# Autodesk Inventor assembly: modularRICH
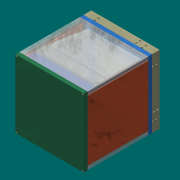
[picture p0: Inventor's stored thumbnail of the model, 180x180]
Saved by Autodesk Inventor 2016 (Build 200138000, 138)
## iProperties
Created: 2015-10-13
Part Number: modularRICH
Document SubType Name: Assembly
Designer: Sawaiz
Author: Sawaiz
## Documents named in this file (8)
- C:\Users\Sawaiz\OneDrive\projects\modularRICH\modularRICH.iam
- C:\Users\Sawaiz\OneDrive\projects\modularRICH\frame\frame.iam
- C:\Users\Sawaiz\OneDrive\projects\modularRICH\aerogelBlock.ipt
- C:\Users\Sawaiz\OneDrive\projects\modularRICH\fresnelLens.ipt
- C:\Users\Sawaiz\OneDrive\projects\modularRICH\mirror\mirrorTopBottom.ipt
- C:\Users\Sawaiz\OneDrive\projects\modularRICH\mirror\mirrorSides.ipt
- C:\Users\Sawaiz\OneDrive\projects\modularRICH\H12700A\H12700A.iam
- C:\Users\Sawaiz\OneDrive\projects\modularRICH\modularRICH.xlsx
## Components (8 placed, 6 different names)
1. frame:1 [sub-assembly] — Mate:1, Flush:1, Mate:3, Angle:4, Mate:4, Mate:5, Mate:6, Mate:7, Mate:8, Mate:9, Mate:10, Mate:11, Mate:12, Mate:13, Mate:14, Mate:15, Flush:3, Flush:4, Mate:16, Mate:17, Flush:5
2. aerogelBlock:1 — Mate:1, Flush:1, Mate:2, Mate:3
3. fresnelLens:1 — Mate:2, Flush:3, Flush:4
4. mirrorSides:1 — Angle:1, Mate:13, Mate:14, Mate:15
5. mirrorSides:2 — Angle:1, Angle:3, Mate:10, Mate:11, Mate:12
6. mirrorTopBottom:3 — Angle:2, Angle:3, Angle:4, Mate:4, Mate:5, Mate:6
7. mirrorTopBottom:4 — Angle:2, Mate:7, Mate:8, Mate:9
8. H12700A:1 [sub-assembly] — Mate:16, Mate:17, Flush:5
## Relationships (25: Mate 17, Flush 4, Angle 4)
- Mate:1: frame:1 ↔ aerogelBlock:1
- Flush:1 (6.35 mm): frame:1 ↔ aerogelBlock:1
- Mate:2: aerogelBlock:1 ↔ fresnelLens:1
- Mate:3: frame:1 ↔ aerogelBlock:1
- Angle:1 (180 deg): mirrorSides:1 ↔ mirrorSides:2
- Angle:2 (180 deg): mirrorTopBottom:3 ↔ mirrorTopBottom:4
- Angle:3 (90 deg): mirrorSides:2 ↔ mirrorTopBottom:3
- Angle:4 (180 deg): frame:1 ↔ mirrorTopBottom:3
- Mate:4: frame:1 ↔ mirrorTopBottom:3
- Mate:5: frame:1 ↔ mirrorTopBottom:3
- Mate:6: frame:1 ↔ mirrorTopBottom:3
- Mate:7: frame:1 ↔ mirrorTopBottom:4
- Mate:8: frame:1 ↔ mirrorTopBottom:4
- Mate:9: frame:1 ↔ mirrorTopBottom:4
- Mate:10: frame:1 ↔ mirrorSides:2
- Mate:11: frame:1 ↔ mirrorSides:2
- Mate:12 (-6.35 mm): frame:1 ↔ mirrorSides:2
- Mate:13: frame:1 ↔ mirrorSides:1
- Mate:14: frame:1 ↔ mirrorSides:1
- Mate:15 (-6.35 mm): frame:1 ↔ mirrorSides:1
- Flush:3 (3.175 mm): frame:1 ↔ fresnelLens:1
- Flush:4 (-3.175 mm): frame:1 ↔ fresnelLens:1
- Mate:16: frame:1 ↔ H12700A:1
- Mate:17: frame:1 ↔ H12700A:1
- Flush:5: frame:1 ↔ H12700A:1
## Named parameters: acrylicThickness = 6.35 mm, aerogelThickness = 20 mm, height = 101.6 mm, width = 101.6 mm, depth = 101.6 mm, mirrorAngle = 5 deg, detectorWidth = 52 mm, detectorHeight = 52 mm, mirrorThickness = 3 mm, fresnelThickness = 0.1 mm, grooveDensity = 100, focalLength = 76.2 mm, ior = 1.49, centerThickness = 1.524 mm, fresnelAngle = 90 deg, fresnelEffectiveDiameter = 76.2 mm, mirrorSuppourtWidth = 38.1 mm, backGrooveBit = 4.8006 mm, sensorHolderWidth = 88.9 mm, sensorHolderSesnorHeight = 53.975 mm, sensorHolderSensorWidth = 53.975 mm, sensorHolderHeight = 88.9 mm, sensorHolderSensorHeight = 53.975 mm, sensorHolderORingGroove = 3.175 mm, sensorHolderORing = 3.175 mm, sensorHolderFlushORingID = 304.8 mm, sensorHolderFlushORing = 3.175 mm, oRingWidth = 3.175 mm, sensorHolderORingID = 203.2 mm, frontBackORingID = 419.1 mm, topBottomHorizontalMirrorGroove = 12.7 mm, backMirrorGroove = 6.35 mm, mirrorGroove = 19.05 mm, compressionPercent = 40, fresnelChamfer = 6.35 mm, mirrorGrooveFillet = 6.35 mm, mirrorGrooveDrill = 6.35 mm, mirrorGrooveMill = 3.175 mm, fresnelMirrorChamfer = 6.35 mm, detectorOpeningHeight = 76.2 mm, detectorOpeningWidth = 76.2 mm
